# Autodesk Inventor assembly: CAM12
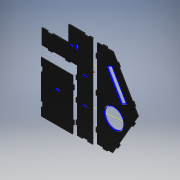
[picture p0: Inventor's stored thumbnail of the model, 180x180]
Saved by Autodesk Inventor 2017 (Build 210142000, 142)
## iProperties
Created: 2019-06-07
Part Number: CAM12
Document SubType Name: Assembly
Designer: Dell
Author: Dell
## Documents named in this file (4)
- C:\Users\Dell\Documents\GitHub\tr2\Body 2.0\CAM12.iam
- C:\Users\Dell\Documents\GitHub\tr2\Body 2.0\BA13.ipt
- C:\Users\Dell\Documents\GitHub\tr2\Body 2.0\BA14.ipt
- C:\Users\Dell\Documents\GitHub\tr2\Body 2.0\BA21.ipt
## Components (3 placed, 3 different names)
1. BA13:1 — Mate:1, Angle:1
2. BA14:1 — Mate:2, Angle:1, Angle:2
3. BA21:1 — Mate:3, Angle:2
## Relationships (5: Mate 3, Angle 2)
- Mate:1: BA13:1
- Mate:2: BA14:1
- Angle:1 (0 deg): BA13:1 ↔ BA14:1
- Mate:3: BA21:1
- Angle:2 (180 deg): BA14:1 ↔ BA21:1
